# Autodesk Inventor assembly: Baugruppe_Crawler
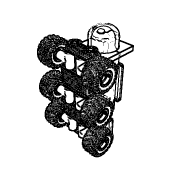
[picture p0: Inventor's stored thumbnail of the model, 180x180]
Saved by Autodesk Inventor 2016 (Build 200138000, 138)
## iProperties
Created: 2015-11-06
Part Number: Baugruppe_Crawler
Document SubType Name: Assembly
Designer: Jonas
Electromechanical_EMX_Project: D:\UNI-Studium\WS_15_16_2. Mastersemester\Marine Robotics\Crawler-Robotic\Kabel.emx
Electromechanical_Physical_Snapshot: D:\UNI-Studium\WS_15_16_2. Mastersemester\Marine Robotics\Crawler-Robotic\Kabel_Physical.snapshot
Electromechanical_Logical_Snapshot: D:\UNI-Studium\WS_15_16_2. Mastersemester\Marine Robotics\Crawler-Robotic\Kabel_Logical.snapshot
Electromechanical_Vault_Folder: EMX\{1C79D629-04D8-4A3A-970E-B5E6892A2958}
_MechatronicsProject: <Project Version="1.0"><Path>D:\UNI-Studium\WS_15_16_2. Mastersemester\Marine Robotics\Crawler-Robotic\Kabel.emx</Path><Guid>{1C79D629-04D8-4A3A-970E-B5E6892A2958}</Guid><IPJFileName>D:\UNI-Studium\WS_15_16_2. Mastersemester\Marine Robotics\Crawler-Robotic\Crawler-Robotik.ipj</IPJFileName><IPJWorkFolder>D:\UNI-Studium\WS_15_16_2. Mastersemester\Marine Robotics\Crawler-Robotic</IPJWorkFolder><AssemblyFileName>D:\UNI-Studium\WS_15_16_2. Mastersemester\Marine Robotics\Crawler-Robotic\Baugruppe_Crawler.iam</AssemblyFileName><AssemblyFileGUID>{9723FAF7-F87D-4BAE-AE12-C84D445CDE3F}</AssemblyFileGUID></Project>
_MTAssemblyInfoProperty: <MechatronicsAssembly Version="1.0" ID="{9723FAF7-F87D-4BAE-AE12-C84D445CDE3F}"><MechatronicsComponents><MechatronicsComponent FileName="switch\lan-femaleconnector.ipt"><ReferenceKey Document="baugruppe_crawler.iam" Value="2|1|1|0|8|0|0|0|23|0|0|0|2|0|0|0|" Context="2|0|0|0|1|0|0|0|" ID="{9723FAF7-F87D-4BAE-AE12-C84D445CDE3F}"/><Properties><ComponentTag>(LAN-FemaleConnector:1)</ComponentTag><TerminalStripTag></TerminalStripTag><TerminalNumberTag></TerminalNumberTag><Installation></Installation><Location></Location><Category></Category><Manufacture></Manufacture><Catalog></Catalog><AssemblyCode></AssemblyCode><Line1></Line1><Line2></Line2><Line3></Line3><ElectricalType></ElectricalType></Properties><OccurrencePath><Occurrence Name="Baugruppe_Steuerung:1" FileName="switch\baugruppe_switch.iam"/><Occurrence Name="LAN-FemaleConnector:1" FileName="switch\lan-femaleconnector.ipt"/></OccurrencePath></MechatronicsComponent><MechatronicsComponent FileName="switch\lan-femaleconnector.ipt"><ReferenceKey Document="baugruppe_crawler.iam" Value="2|1|1|0|8|0|0|0|23|0|0|0|3|0|0|0|" Context="2|0|0|0|1|0|0|0|" ID="{9723FAF7-F87D-4BAE-AE12-C84D445CDE3F}"/><Properties><ComponentTag>(LAN-FemaleConnector:2)</ComponentTag><TerminalStripTag></TerminalStripTag><TerminalNumberTag></TerminalNumberTag><Installation></Installation><Location></Location><Category></Category><Manufacture></Manufacture><Catalog></Catalog><AssemblyCode></AssemblyCode><Line1></Line1><Line2></Line2><Line3></Line3><ElectricalType></ElectricalType></Properties><OccurrencePath><Occurrence Name="Baugruppe_Steuerung:1" FileName="switch\baugruppe_switch.iam"/><Occurrence Name="LAN-FemaleConnector:2" FileName="switch\lan-femaleconnector.ipt"/></OccurrencePath></MechatronicsComponent><MechatronicsComponent FileName="switch\lan-femaleconnector.ipt"><ReferenceKey Document="baugruppe_crawler.iam" Value="2|1|1|0|8|0|0|0|23|0|0|0|4|0|0|0|" Context="2|0|0|0|1|0|0|0|" ID="{9723FAF7-F87D-4BAE-AE12-C84D445CDE3F}"/><Properties><ComponentTag>(LAN-FemaleConnector:3)</ComponentTag><TerminalStripTag></TerminalStripTag><TerminalNumberTag></TerminalNumberTag><Installation></Installation><Location></Location><Category></Category><Manufacture></Manufacture><Catalog></Catalog><AssemblyCode></AssemblyCode><Line1></Line1><Line2></Line2><Line3></Line3><ElectricalType></ElectricalType></Properties><OccurrencePath><Occurrence Name="Baugruppe_Steuerung:1" FileName="switch\baugruppe_switch.iam"/><Occurrence Name="LAN-FemaleConnector:3" FileName="switch\lan-femaleconnector.ipt"/></OccurrencePath></MechatronicsComponent><MechatronicsComponent FileName="switch\lan-femaleconnector.ipt"><ReferenceKey Document="baugruppe_crawler.iam" Value="2|1|1|0|8|0|0|0|23|0|0|0|5|0|0|0|" Context="2|0|0|0|1|0|0|0|" ID="{9723FAF7-F87D-4BAE-AE12-C84D445CDE3F}"/><Properties><ComponentTag>(LAN-FemaleConnector:4)</ComponentTag><TerminalStripTag></TerminalStripTag><TerminalNumberTag></TerminalNumberTag><Installation></Installation><Location></Location><Category></Category><Manufacture></Manufacture><Catalog></Catalog><AssemblyCode></AssemblyCode><Line1></Line1><Line2></Line2><Line3></Line3><ElectricalType></ElectricalType></Properties><OccurrencePath><Occurrence Name="Baugruppe_Steuerung:1" FileName="switch\baugruppe_switch.iam"/><Occurrence Name="LAN-FemaleConnector:4" FileName="switch\lan-femaleconnector.ipt"/></OccurrencePath></MechatronicsComponent><MechatronicsComponent FileName="switch\lan-femaleconnector.ipt"><ReferenceKey Document="baugruppe_crawler.iam" Value="2|1|1|0|8|0|0|0|23|0|0|0|6|0|0|0|" Context="2|0|0|0|1|0|0|0|" ID="{9723FAF7-F87D-4BAE-AE12-C84D445CDE3F}"/><Properties><ComponentTag>(LAN-FemaleConnector:5)</ComponentTag><TerminalStripTag></TerminalStripTag><TerminalNumberTag></TerminalNumberTag><Installation></Installation><Location></Location><Category></Category><Manufacture></Manufacture><Catalog></Catalog><AssemblyCode></AssemblyCode><Line1></Line1><Line2></Line2><Line3></Line3><ElectricalType></ElectricalType></Properties><OccurrencePath><Occurrence Name="Baugruppe_Steuerung:1" FileName="switch\baugruppe_switch.iam"/><Occurrence Name="LAN-FemaleConnector:5" FileName="switch\lan-femaleconnector.ipt"/></OccurrencePath></MechatronicsComponent><MechatronicsComponent FileName="beagleboneblack\beagleboneblack.ipt"><ReferenceKey Document="baugruppe_crawler.iam" Value="2|1|1|0|8|0|0|0|23|0|0|0|9|0|0|0|" Context="2|0|0|0|1|0|0|0|" ID="{9723FAF7-F87D-4BAE-AE12-C84D445CDE3F}"/><Properties><ComponentTag>(BeagleboneBlack:1)</ComponentTag><TerminalStripTag></TerminalStripTag><TerminalNumberTag></TerminalNumberTag><Installation></Installation><Location></Location><Category></Category><Manufacture></Manufacture><Catalog></Catalog><AssemblyCode></AssemblyCode><Line1></Line1><Line2></Line2><Line3></Line3><ElectricalType></ElectricalType></Properties><OccurrencePath><Occurrence Name="Baugruppe_Steuerung:1" FileName="switch\baugruppe_switch.iam"/><Occurrence Name="BeagleboneBlack:1" FileName="beagleboneblack\beagleboneblack.ipt"/></OccurrencePath></MechatronicsComponent><MechatronicsComponent FileName="battery\akkublock.ipt"><ReferenceKey Document="baugruppe_crawler.iam" Value="2|1|1|0|8|0|0|0|24|0|0|0|1|0|0|0|" Context="2|0|0|0|1|0|0|0|" ID="{9723FAF7-F87D-4BAE-AE12-C84D445CDE3F}"/><Properties><ComponentTag>(Akkublock:1)</ComponentTag><TerminalStripTag></TerminalStripTag><TerminalNumberTag></TerminalNumberTag><Installation></Installation><Location></Location><Category></Category><Manufacture></Manufacture><Catalog></Catalog><AssemblyCode></AssemblyCode><Line1></Line1><Line2></Line2><Line3></Line3><ElectricalType></ElectricalType></Properties><OccurrencePath><Occurrence Name="Baugruppe_Akku:1" FileName="battery\baugruppe_akku.iam"/><Occurrence Name="Akkublock:1" FileName="battery\akkublock.ipt"/></OccurrencePath></MechatronicsComponent><MechatronicsComponent FileName="battery\akkublock.ipt"><ReferenceKey Document="baugruppe_crawler.iam" Value="2|1|1|0|8|0|0|0|24|0|0|0|3|0|0|0|" Context="2|0|0|0|1|0|0|0|" ID="{9723FAF7-F87D-4BAE-AE12-C84D445CDE3F}"/><Properties><ComponentTag>(Akkublock:2)</ComponentTag><TerminalStripTag></TerminalStripTag><TerminalNumberTag></TerminalNumberTag><Installation></Installation><Location></Location><Category></Category><Manufacture></Manufacture><Catalog></Catalog><AssemblyCode></AssemblyCode><Line1></Line1><Line2></Line2><Line3></Line3><ElectricalType></ElectricalType></Properties><OccurrencePath><Occurrence Name="Baugruppe_Akku:1" FileName="battery\baugruppe_akku.iam"/><Occurrence Name="Akkublock:2" FileName="battery\akkublock.ipt"/></OccurrencePath></MechatronicsComponent></MechatronicsComponents><MechatronicsComponentDefs><MechatronicsComponentDef DocInternalName="{ACCBE6A6-47E8-CFEC-FC20-359788D8907B}" FileName="switch\lan-femaleconnector.ipt" DocRevID="{56A72F35-41BF-9B6B-30B7-3CBA8042FC9F}" iPropertyRevID="{4A98FA15-FCEF-403A-97C5-5A6B14D3200A}"><Pins><Pin PinIndex="1" PinName="1"/><Pin PinIndex="2" PinName="2"/></Pins></MechatronicsComponentDef><MechatronicsComponentDef DocInternalName="{C815D725-4DF9-D355-EAFB-AD84FE3D8762}" FileName="beagleboneblack\beagleboneblack.ipt" DocRevID="{BBD8A078-4D52-5844-0310-229E39F81467}" iPropertyRevID="{AC44C654-C93A-4CFF-BA6B-6D45999ECA81}"><Pins><Pin PinIndex="1" PinName="1"/><Pin PinIndex="2" PinName="2"/><Pin PinIndex="3" PinName="3"/><Pin PinIndex="4" PinName="4"/></Pins></MechatronicsComponentDef><MechatronicsComponentDef DocInternalName="{3A56D286-4DDC-642B-E8B2-688C9AF892F2}" FileName="battery\akkublock.ipt" DocRevID="{85B8ECE5-4815-0560-3E8D-A48C5999F7C5}" iPropertyRevID="{6B78ED58-7F91-4AD7-96AF-31CC6D480C74}"><Pins><Pin PinIndex="1" PinName="1"/><Pin PinIndex="2" PinName="2"/></Pins></MechatronicsComponentDef></MechatronicsComponentDefs><MechatronicsHarnessAssemblies/><MechatronicsConnectionDefs/><MechatronicsConnections/><MechatronicsCableDefs/><MechatronicsCables/><MechatronicsSubAssemblies/><ComponentLinks/><MechatronicsAssemblyRevision FileRevision="46"><Occurrences><Occurrence FileName="C:\Users\Andreas\Documents\Inventor\Content Center Files\R2016\de-DE\DIN 7985 (Z)\DIN 7985 (Z) - M3x8-Z.ipt" Name="DIN 7985 (Z) M3x8-Z:1" FileRevision="{7EEA30AF-53F6-0C49-D56E-7E6FA6F3236C}"/><Occurrence FileName="C:\Users\Andreas\Documents\Inventor\Content Center Files\R2016\de-DE\DIN 7985 (Z)\DIN 7985 (Z) - M3x8-Z.ipt" Name="DIN 7985 (Z) M3x8-Z:2" FileRevision="{7EEA30AF-53F6-0C49-D56E-7E6FA6F3236C}"/><Occurrence FileName="arexx-chassie\baugruppe_arexx-chassie.iam" Name="Baugruppe_AREXX-Chassie:1" FileRevision="{1AA6BBCA-9950-7C2D-DF1B-7E7C464C9497}"/><Occurrence FileName="battery\baugruppe_akku.iam" Name="Baugruppe_Akku:1" FileRevision="{9B1FE8EA-8753-26D1-4D09-1AFA0104BB93}"/><Occurrence FileName="buchsen_un_stecker\rohr_controller_motor.ipt" Name="Rohr_Controller_Motor:1" FileRevision="{56151D24-1544-1A9A-CFDC-32BB28AA60E5}"/><Occurrence FileName="led\baugruppe_led.iam" Name="Baugruppe_LED:1" FileRevision="{03D59B67-AE27-9444-9279-69A09F1D7551}"/><Occurrence FileName="led\baugruppe_led.iam" Name="Baugruppe_LED:2" FileRevision="{03D59B67-AE27-9444-9279-69A09F1D7551}"/><Occurrence FileName="motordriver_pololu\baugruppe_motordriver_housing.iam" Name="Baugruppe_Motordriver_Housing:1" FileRevision="{086E4759-0B4B-FD0D-00EB-DCAA3B3E223C}"/><Occurrence FileName="sricam\baugruppe_camera.iam" Name="Baugruppe_Camera:1" FileRevision="{A461D180-9B9F-CDAE-AB06-8E7A994C6AD4}"/><Occurrence FileName="switch\baugruppe_switch.iam" Name="Baugruppe_Steuerung:1" FileRevision="{D45E2017-CCCA-7F8B-5D45-0C8411629959}"/></Occurrences></MechatronicsAssemblyRevision></MechatronicsAssembly>
Author: Jonas
## Documents named in this file (9)
- D:\UNI-Studium\WS_15_16_2. Mastersemester\Marine Robotics\Crawler-Robotic\Baugruppe_Crawler.iam
- D:\UNI-Studium\WS_15_16_2. Mastersemester\Marine Robotics\Crawler-Robotic\AREXX-Chassie\Baugruppe_AREXX-Chassie.iam
- D:\UNI-Studium\WS_15_16_2. Mastersemester\Marine Robotics\Crawler-Robotic\Sricam\Baugruppe_Camera.iam
- D:\UNI-Studium\WS_15_16_2. Mastersemester\Marine Robotics\Crawler-Robotic\Motordriver_Pololu\Baugruppe_Motordriver_Housing.iam
- D:\UNI-Studium\WS_15_16_2. Mastersemester\Marine Robotics\Crawler-Robotic\Switch\Baugruppe_Switch.iam
- D:\UNI-Studium\WS_15_16_2. Mastersemester\Marine Robotics\Crawler-Robotic\Battery\Baugruppe_Akku.iam
- D:\UNI-Studium\WS_15_16_2. Mastersemester\Marine Robotics\Crawler-Robotic\Buchsen_un_Stecker\Rohr_Controller_Motor.ipt
- C:\Users\Andreas\Documents\Inventor\Content Center Files\R2016\de-DE\DIN 7985 (Z)\DIN 7985 (Z) - M3x8-Z.ipt
- D:\UNI-Studium\WS_15_16_2. Mastersemester\Marine Robotics\Crawler-Robotic\LED\Baugruppe_LED.iam
## Components (10 placed, 8 different names)
1. Baugruppe_AREXX-Chassie:1 [sub-assembly] — Passend:6, Passend:9, Fluchtend:4, Passend:11, Einfügen:3, Einfügen:4, Einfügen:5, Einfügen:6, Einfügen:7, Einfügen:8, Winkel:1
2. Baugruppe_Camera:1 [sub-assembly] — Einfügen:3, Einfügen:4
3. Baugruppe_Motordriver_Housing:1 [sub-assembly] — Passend:6, Einfügen:2
4. Baugruppe_Steuerung:1 [sub-assembly] — Passend:9, Fluchtend:4, Passend:12, Fluchtend:5, Fluchtend:6, Einfügen:1
5. Baugruppe_Akku:1 [sub-assembly] — Passend:12, Fluchtend:5, Fluchtend:6
6. Rohr_Controller_Motor:1 — Einfügen:1, Einfügen:2
7. DIN 7985 (Z) M3x8-Z:1 — Einfügen:6
8. DIN 7985 (Z) M3x8-Z:2 — Einfügen:5
9. Baugruppe_LED:1 [sub-assembly] — Einfügen:8, Winkel:2
10. Baugruppe_LED:2 [sub-assembly] — Einfügen:7, Winkel:1
## Relationships (17: Insert 8, Mate 4, Flush 3, Angle 2)
- Passend:6 [Mate]: Baugruppe_AREXX-Chassie:1 ↔ Baugruppe_Motordriver_Housing:1
- Passend:9 [Mate]: Baugruppe_AREXX-Chassie:1 ↔ Baugruppe_Steuerung:1
- Fluchtend:4 [Flush] (2 mm): Baugruppe_AREXX-Chassie:1 ↔ Baugruppe_Steuerung:1
- Passend:11 [Mate]: Baugruppe_AREXX-Chassie:1
- Passend:12 [Mate]: Baugruppe_Steuerung:1 ↔ Baugruppe_Akku:1
- Fluchtend:5 [Flush] (10 mm): Baugruppe_Steuerung:1 ↔ Baugruppe_Akku:1
- Fluchtend:6 [Flush] (10 mm): Baugruppe_Steuerung:1 ↔ Baugruppe_Akku:1
- Einfügen:1 [Insert]: Baugruppe_Steuerung:1 ↔ Rohr_Controller_Motor:1
- Einfügen:2 [Insert]: Baugruppe_Motordriver_Housing:1 ↔ Rohr_Controller_Motor:1
- Einfügen:3 [Insert]: Baugruppe_AREXX-Chassie:1 ↔ Baugruppe_Camera:1
- Einfügen:4 [Insert]: Baugruppe_AREXX-Chassie:1 ↔ Baugruppe_Camera:1
- Einfügen:5 [Insert]: Baugruppe_AREXX-Chassie:1 ↔ DIN 7985 (Z) M3x8-Z:2
- Einfügen:6 [Insert]: Baugruppe_AREXX-Chassie:1 ↔ DIN 7985 (Z) M3x8-Z:1
- Einfügen:7 [Insert]: Baugruppe_AREXX-Chassie:1 ↔ Baugruppe_LED:2
- Einfügen:8 [Insert]: Baugruppe_AREXX-Chassie:1 ↔ Baugruppe_LED:1
- Winkel:1 [Angle] (180 deg): Baugruppe_AREXX-Chassie:1 ↔ Baugruppe_LED:2
- Winkel:2 [Angle] (0 deg): Baugruppe_LED:1
